# Autodesk Inventor assembly: Viewpoint
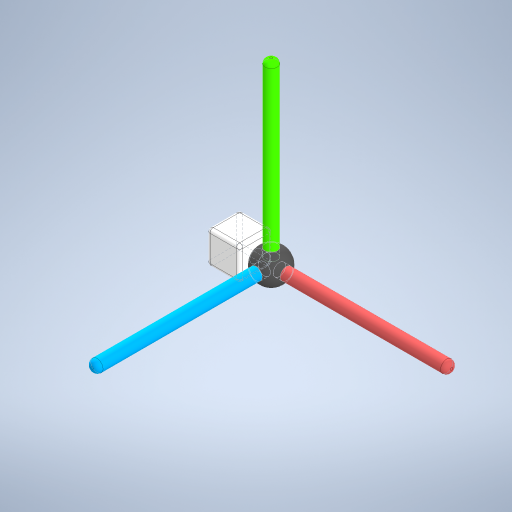
[picture p0: Inventor's stored thumbnail of the model, 512x512]
Saved by Autodesk Inventor 2023 (Build 270158000, 158)
## iProperties
Created: 2022-12-13
Part Number: Viewpoint
Document SubType Name: Assembly
Designer: romanp
Author: romanp
## Documents named in this file (4)
- C:\Users\romanp\Desktop\Viewpoint.iam
- C:\Users\romanp\Desktop\Line.ipt
- C:\Users\romanp\Desktop\Base2.ipt
- C:\Users\romanp\Desktop\Holder.ipt
## Components (5 placed, 3 different names)
1. Line:3 — Insert:1
2. Base:1 — Insert:1, Insert:3, Insert:5, Insert:6
3. Line:5 — Insert:3
4. Line:6 — Insert:5
5. Holder:1 — Insert:6
## Relationships (4: Insert 4)
- Insert:1: Line:3 ↔ Base:1
- Insert:3: Base:1 ↔ Line:5
- Insert:5: Base:1 ↔ Line:6
- Insert:6: Base:1 ↔ Holder:1
